# Autodesk Inventor assembly: Сборка
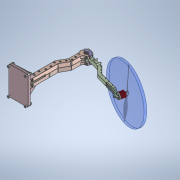
[picture p0: Inventor's stored thumbnail of the model, 180x180]
Saved by Autodesk Inventor 2021.2 (Build 252289000, 289)
## iProperties
Created: 2024-10-29
Part Number: Сборка
Document SubType Name: Assembly
Designer: barko
Mass: 1383.59 g
Surface Area: 2828.64 cm^2
Volume: 1218.78 cm^3
Density: 1.13522 g/cm^3
Author: barko
## Documents named in this file (31)
- C:\Users\DELL\Desktop\Personal\PID_controller\PID_controller\Mechanics\3D_model\Сборка.iam
- C:\Users\DELL\Desktop\Personal\PID_controller\PID_controller\Mechanics\3D_model\Детали твёрдого тела\Скобка 1.ipt
- C:\Users\DELL\Desktop\Personal\PID_controller\PID_controller\Mechanics\3D_model\Детали твёрдого тела\Скобка 2.ipt
- C:\Users\DELL\Desktop\Personal\PID_controller\PID_controller\Mechanics\3D_model\Детали твёрдого тела\Фланец.ipt
- C:\Users\DELL\Desktop\Personal\PID_controller\PID_controller\Mechanics\3D_model\Детали твёрдого тела\Луч.ipt
- C:\Users\DELL\Desktop\Personal\PID_controller\PID_controller\Mechanics\3D_model\Детали твёрдого тела\Ложечка.ipt
- C:\Users\DELL\Desktop\Personal\PID_controller\PID_controller\Mechanics\3D_model\Моторчик.ipt
- C:\Users\DELL\Desktop\Personal\PID_controller\PID_controller\Mechanics\3D_model\Пропеллер.ipt
- C:\Users\DELL\Documents\Inventor\Content Center Files\R2021\ru-RU\Nut GOST 15524-70\Гайка M4-6H ГОСТ 15524-70.ipt
- C:\Users\DELL\Documents\Inventor\Content Center Files\R2021\ru-RU\GOST 11738-84\Винт M4-6gx20 ГОСТ 11738-84.ipt
- C:\Users\DELL\Desktop\Personal\PID_controller\PID_controller\Mechanics\3D_model\Подшипник.ipt
- C:\Users\DELL\Documents\Inventor\Content Center Files\R2021\ru-RU\GOST 5915-70\Гайка M6-6H ГОСТ 5915-70(1).ipt
- C:\Users\DELL\Documents\Inventor\Content Center Files\R2021\ru-RU\GOST 11738-84\Винт M6-6gx50 ГОСТ 11738-84.ipt
- C:\Users\DELL\Documents\Inventor\Content Center Files\R2021\ru-RU\GOST 11371-78  A\Шайба 6 ГОСТ 11371-78.ipt
- C:\Users\DELL\Documents\Inventor\Content Center Files\R2021\ru-RU\Washer 1 GOST 6402-78\Шайба 6Л ГОСТ 6402-78.ipt
- C:\Users\DELL\Documents\Inventor\Content Center Files\R2021\ru-RU\GOST 17475-80 (2)\Винт 2.M6-6gx30 ГОСТ 17475-80.ipt
- C:\Users\DELL\Documents\Inventor\Content Center Files\R2021\ru-RU\ISO 10642(1)\ISO 10642 - M3x8.ipt
- C:\Users\DELL\Documents\Inventor\Content Center Files\R2021\ru-RU\ISO 10642(1)\ISO 10642 - M3x12.ipt
- C:\Users\DELL\Desktop\Personal\PID_controller\PID_controller\Mechanics\3D_model\Детали твёрдого тела\Вал насадка 1.ipt
- C:\Users\DELL\Desktop\Personal\PID_controller\PID_controller\Mechanics\3D_model\Метизы\Шайба A 4 ГОСТ 6958-78.ipt
- C:\Users\DELL\Documents\Inventor\Content Center Files\R2021\ru-RU\GOST 5916-70\Гайка M4-6H ГОСТ 5916-70.ipt
- C:\Users\DELL\Documents\Inventor\Content Center Files\R2021\ru-RU\GOST 11738-84\Винт M4-6gx25 ГОСТ 11738-84.ipt
- C:\Users\DELL\Documents\Inventor\Content Center Files\R2021\ru-RU\GOST 11738-84\Винт M6-6gx30 ГОСТ 11738-84.ipt
- C:\Users\DELL\Desktop\Personal\PID_controller\PID_controller\Mechanics\3D_model\Детали твёрдого тела\Блок.ipt
- C:\Users\DELL\Desktop\Personal\PID_controller\PID_controller\Mechanics\3D_model\Детали твёрдого тела\Ножка левая верх.ipt
- C:\Users\DELL\Desktop\Personal\PID_controller\PID_controller\Mechanics\3D_model\Детали твёрдого тела\Ножка левая низ.ipt
- C:\Users\DELL\Desktop\Personal\PID_controller\PID_controller\Mechanics\3D_model\Детали твёрдого тела\Ножка правая верх.ipt
- C:\Users\DELL\Desktop\Personal\PID_controller\PID_controller\Mechanics\3D_model\Детали твёрдого тела\Ножка правая низ.ipt
- C:\Users\DELL\Documents\Inventor\Content Center Files\R2021\ru-RU\GOST 11738-84\Винт M4-6gx30 ГОСТ 11738-84.ipt
- C:\Users\DELL\Desktop\Personal\PID_controller\PID_controller\Mechanics\3D_model\Метизы\Винт M3-6gx8 ГОСТ 11738-84.ipt
- C:\Users\DELL\Desktop\Personal\PID_controller\PID_controller\Mechanics\3D_model\Метизы\Винт M4-6gx40 ГОСТ 1491-80.ipt
## Components (78 placed, 30 different names)
1. Скобка 1:1 — Совмещение:104, Совмещение:109
2. Скобка 2:1 — Совмещение:119, Совмещение:120
3. Фланец:1 — Вставка:6, Вставка:7, Вставка:8, Вставка:9, Заподлицо:2, Заподлицо:3, Заподлицо:4, Заподлицо:5, Совмещение:127, Совмещение:128, Совмещение:129, Совмещение:130, Совмещение:131, Совмещение:132, Совмещение:133, Совмещение:134, Совмещение:135, Совмещение:136, Совмещение:137, Совмещение:138
4. Луч:1 — Заподлицо:1, Совмещение:96, Совмещение:97, Заподлицо:6, Совмещение:111, Совмещение:112, Совмещение:114, Совмещение:199
5. Ложечка:1 — Совмещение:87, Совмещение:88, Совмещение:91, Совмещение:92, Совмещение:93, Совмещение:94, Совмещение:96, Совмещение:97, Заподлицо:6, Совмещение:98, Совмещение:99, Вставка:37
6. Моторчик:1 — Вставка:2, Совмещение:98, Совмещение:99
7. Пропеллер:1 — Вставка:2
8. Подшипник:1 — Вставка:25, Вставка:29, Вставка:39
9. Подшипник:2 — Вставка:32, Вставка:34
10. Вал насадка 1:1 — Вставка:25, Вставка:32, Совмещение:199
11. Шайба A 4 ГОСТ 6958-78:3 — Вставка:29, Вставка:38
12. Блок:1
13. Шайба A 4 ГОСТ 6958-78:4 — Вставка:34, Вставка:36
14. Гайка ГОСТ 15524-70 M4:7 — Вставка:36
15. Ножка левая верх:1 — Совмещение:152, Совмещение:153, Совмещение:154, Совмещение:155, Совмещение:156, Совмещение:157, Совмещение:213, Совмещение:215, Совмещение:231, Совмещение:233, Совмещение:235, Совмещение:237, Совмещение:239, Совмещение:241, Совмещение:243
16. Ножка левая низ:1 — Совмещение:143, Совмещение:145
17. Ножка правая верх:1 — Совмещение:147, Совмещение:148, Совмещение:149, Совмещение:150, Совмещение:151, Совмещение:158, Вставка:39, Совмещение:208, Совмещение:209, Совмещение:210, Совмещение:211, Совмещение:212, Совмещение:214
18. Ножка правая низ:1 — Совмещение:144, Совмещение:146, Совмещение:216, Совмещение:217, Совмещение:218, Совмещение:219, Совмещение:220, Совмещение:221, Совмещение:222, Совмещение:223, Совмещение:224, Совмещение:225, Совмещение:226, Совмещение:227, Совмещение:228, Совмещение:229, Совмещение:230, Совмещение:232, Совмещение:234, Совмещение:236, Совмещение:238, Совмещение:240, Совмещение:242
19. Винт M4-6gx40 ГОСТ 1491-80:1 — Вставка:38
20. Винт ГОСТ 11738-84 M 4x30:4 — Совмещение:216, Совмещение:217
21. Гайка ГОСТ 5916-70 M4:4 — Совмещение:230, Совмещение:231
22. Винт ГОСТ 11738-84 M 4x30:6 — Совмещение:218, Совмещение:219
23. Винт ГОСТ 11738-84 M 4x30:7 — Совмещение:220, Совмещение:221
24. Винт ГОСТ 11738-84 M 4x30:8 — Совмещение:222, Совмещение:223
25. Винт ГОСТ 11738-84 M 4x30:9 — Совмещение:224, Совмещение:225
26. Винт ГОСТ 11738-84 M 4x30:10 — Совмещение:226, Совмещение:227
27. Винт ГОСТ 11738-84 M 4x30:11 — Совмещение:228, Совмещение:229
28. Гайка ГОСТ 5916-70 M4:6 — Совмещение:232, Совмещение:233
29. Гайка ГОСТ 5916-70 M4:7 — Совмещение:234, Совмещение:235
30. Гайка ГОСТ 5916-70 M4:8 — Совмещение:236, Совмещение:237
31. Гайка ГОСТ 5916-70 M4:9 — Совмещение:238, Совмещение:239
32. Гайка ГОСТ 5916-70 M4:10 — Совмещение:240, Совмещение:241
33. Гайка ГОСТ 5916-70 M4:11 — Совмещение:242, Совмещение:243
34. Гайка ГОСТ 5916-70 M4:5 — Совмещение:214, Совмещение:215
35. Винт ГОСТ 11738-84 M 4x30:5 — Совмещение:210, Совмещение:211
36. Гайка ГОСТ 5916-70 M4:1 — Совмещение:212, Совмещение:213
37. Винт ГОСТ 11738-84 M 4x30:1 — Совмещение:208, Совмещение:209
38. Винт ГОСТ 11738-84 M 4x25:1 — Совмещение:103, Совмещение:104
39. Гайка ГОСТ 15524-70 M4:1 — Совмещение:103, Совмещение:147, Совмещение:148, Совмещение:149
40. Винт ГОСТ 11738-84 M 4x25:2 — Совмещение:113, Совмещение:114
41. Гайка ГОСТ 15524-70 M4:2 — Совмещение:111, Совмещение:112, Совмещение:113
42. Винт ГОСТ 11738-84 M 4x20:2 — Совмещение:108, Совмещение:109
43. Винт ГОСТ 11738-84 M 4x25:3 — Совмещение:118, Совмещение:119
44. Винт ГОСТ 11738-84 M 4x20:4 — Совмещение:120, Совмещение:124
45. Гайка ГОСТ 15524-70 M4:3 — Совмещение:118, Совмещение:155, Совмещение:156, Совмещение:157
46. Гайка ГОСТ 15524-70 M4:4 — Совмещение:108, Совмещение:150, Совмещение:151, Совмещение:158
47. Гайка ГОСТ 15524-70 M4:5 — Совмещение:124, Совмещение:152, Совмещение:153, Совмещение:154
48. Гайка ГОСТ 5915-70 M6:1 — Совмещение:133, Совмещение:134, Совмещение:135, Совмещение:140
49. Гайка ГОСТ 5915-70 M6:2 — Совмещение:127, Совмещение:128, Совмещение:129, Совмещение:139
50. Гайка ГОСТ 5915-70 M6:3 — Совмещение:136, Совмещение:137, Совмещение:138, Совмещение:141
51. Гайка ГОСТ 5915-70 M6:4 — Совмещение:78, Совмещение:130, Совмещение:131, Совмещение:132, Совмещение:142
52. Винт ГОСТ 11738-84 M 6x50:1 — Совмещение:141, Совмещение:146
53. Винт ГОСТ 11738-84 M 6x30:1 — Совмещение:139, Совмещение:143
54. Винт ГОСТ 11738-84 M 6x30:2 — Совмещение:78, Совмещение:142, Совмещение:144
55. Винт ГОСТ 11738-84 M 6x50:2 — Совмещение:140, Совмещение:145
56. Шайба  ГОСТ 11371-78 6,4:1 — Вставка:6, Вставка:10
57. Шайба  ГОСТ 11371-78 6,4:2 — Вставка:7, Вставка:11
58. Шайба  ГОСТ 11371-78 6,4:3 — Вставка:8, Вставка:13
59. Шайба  ГОСТ 11371-78 6,4:4 — Вставка:9, Вставка:12
60. Шайба 1 ГОСТ 6402-78 6Л:1 — Вставка:10, Вставка:16
61. Шайба 1 ГОСТ 6402-78 6Л:2 — Вставка:11, Вставка:15
62. Шайба 1 ГОСТ 6402-78 6Л:3 — Вставка:12, Вставка:17
63. Шайба 1 ГОСТ 6402-78 6Л:4 — Вставка:13, Вставка:14
64. Гайка ГОСТ 5915-70 M6:5 — Вставка:14, Совмещение:85
65. Гайка ГОСТ 5915-70 M6:6 — Вставка:15, Совмещение:84
66. Гайка ГОСТ 5915-70 M6:7 — Вставка:16, Совмещение:82
67. Гайка ГОСТ 5915-70 M6:8 — Вставка:17, Совмещение:83
68. Винт 2 ГОСТ 17475-80 M6 x 30:1 — Совмещение:82, Заподлицо:3
69. Винт 2 ГОСТ 17475-80 M6 x 30:2 — Совмещение:83, Заподлицо:2
70. Винт 2 ГОСТ 17475-80 M6 x 30:3 — Совмещение:85, Заподлицо:5
71. Винт 2 ГОСТ 17475-80 M6 x 30:4 — Совмещение:84, Заподлицо:4
72. Винт M3-6gx8 ГОСТ 11738-84:1 — Вставка:37
73. ISO 10642 M3x12:2 — Совмещение:87
74. ISO 10642 M3x12:3 — Совмещение:88
75. ISO 10642 M3x8:1 — Совмещение:91
76. ISO 10642 M3x8:2 — Совмещение:92
77. ISO 10642 M3x8:3 — Совмещение:93
78. ISO 10642 M3x8:4 — Совмещение:94
## Relationships (123: Mate 96, Insert 21, Flush 6)
- Вставка:2 [Insert] (2 mm): Моторчик:1 ↔ Пропеллер:1
- Заподлицо:1 [Flush]: Луч:1
- Совмещение:78 [Mate]: Гайка ГОСТ 5915-70 M6:4 ↔ Винт ГОСТ 11738-84 M 6x30:2
- Вставка:6 [Insert]: Фланец:1 ↔ Шайба  ГОСТ 11371-78 6,4:1
- Вставка:7 [Insert]: Фланец:1 ↔ Шайба  ГОСТ 11371-78 6,4:2
- Вставка:8 [Insert]: Фланец:1 ↔ Шайба  ГОСТ 11371-78 6,4:3
- Вставка:9 [Insert]: Фланец:1 ↔ Шайба  ГОСТ 11371-78 6,4:4
- Вставка:10 [Insert]: Шайба  ГОСТ 11371-78 6,4:1 ↔ Шайба 1 ГОСТ 6402-78 6Л:1
- Вставка:11 [Insert]: Шайба  ГОСТ 11371-78 6,4:2 ↔ Шайба 1 ГОСТ 6402-78 6Л:2
- Вставка:12 [Insert]: Шайба  ГОСТ 11371-78 6,4:4 ↔ Шайба 1 ГОСТ 6402-78 6Л:3
- Вставка:13 [Insert]: Шайба  ГОСТ 11371-78 6,4:3 ↔ Шайба 1 ГОСТ 6402-78 6Л:4
- Вставка:14 [Insert]: Шайба 1 ГОСТ 6402-78 6Л:4 ↔ Гайка ГОСТ 5915-70 M6:5
- Вставка:15 [Insert]: Шайба 1 ГОСТ 6402-78 6Л:2 ↔ Гайка ГОСТ 5915-70 M6:6
- Вставка:16 [Insert]: Шайба 1 ГОСТ 6402-78 6Л:1 ↔ Гайка ГОСТ 5915-70 M6:7
- Вставка:17 [Insert]: Шайба 1 ГОСТ 6402-78 6Л:3 ↔ Гайка ГОСТ 5915-70 M6:8
- Совмещение:82 [Mate]: Гайка ГОСТ 5915-70 M6:7 ↔ Винт 2 ГОСТ 17475-80 M6 x 30:1
- Совмещение:83 [Mate]: Гайка ГОСТ 5915-70 M6:8 ↔ Винт 2 ГОСТ 17475-80 M6 x 30:2
- Совмещение:84 [Mate]: Гайка ГОСТ 5915-70 M6:6 ↔ Винт 2 ГОСТ 17475-80 M6 x 30:4
- Совмещение:85 [Mate]: Гайка ГОСТ 5915-70 M6:5 ↔ Винт 2 ГОСТ 17475-80 M6 x 30:3
- Заподлицо:2 [Flush] (9 mm): Фланец:1 ↔ Винт 2 ГОСТ 17475-80 M6 x 30:2
- Заподлицо:3 [Flush] (9 mm): Фланец:1 ↔ Винт 2 ГОСТ 17475-80 M6 x 30:1
- Заподлицо:4 [Flush] (9 mm): Фланец:1 ↔ Винт 2 ГОСТ 17475-80 M6 x 30:4
- Заподлицо:5 [Flush] (9 mm): Фланец:1 ↔ Винт 2 ГОСТ 17475-80 M6 x 30:3
- Совмещение:87 [Mate]: Ложечка:1 ↔ ISO 10642 M3x12:2
- Совмещение:88 [Mate]: Ложечка:1 ↔ ISO 10642 M3x12:3
- Совмещение:91 [Mate]: Ложечка:1 ↔ ISO 10642 M3x8:1
- Совмещение:92 [Mate]: Ложечка:1 ↔ ISO 10642 M3x8:2
- Совмещение:93 [Mate]: Ложечка:1 ↔ ISO 10642 M3x8:3
- Совмещение:94 [Mate]: Ложечка:1 ↔ ISO 10642 M3x8:4
- Совмещение:96 [Mate]: Луч:1 ↔ Ложечка:1
- Совмещение:97 [Mate]: Луч:1 ↔ Ложечка:1
- Заподлицо:6 [Flush]: Луч:1 ↔ Ложечка:1
- Совмещение:98 [Mate]: Ложечка:1 ↔ Моторчик:1
- Совмещение:99 [Mate]: Ложечка:1 ↔ Моторчик:1
- Вставка:25 [Insert]: Подшипник:1 ↔ Вал насадка 1:1
- Совмещение:103 [Mate]: Винт ГОСТ 11738-84 M 4x25:1 ↔ Гайка ГОСТ 15524-70 M4:1
- Совмещение:104 [Mate]: Скобка 1:1 ↔ Винт ГОСТ 11738-84 M 4x25:1
- Совмещение:108 [Mate]: Винт ГОСТ 11738-84 M 4x20:2 ↔ Гайка ГОСТ 15524-70 M4:4
- Совмещение:109 [Mate]: Скобка 1:1 ↔ Винт ГОСТ 11738-84 M 4x20:2
- Совмещение:111 [Mate]: Луч:1 ↔ Гайка ГОСТ 15524-70 M4:2
- Совмещение:112 [Mate]: Луч:1 ↔ Гайка ГОСТ 15524-70 M4:2
- Совмещение:113 [Mate]: Винт ГОСТ 11738-84 M 4x25:2 ↔ Гайка ГОСТ 15524-70 M4:2
- Совмещение:114 [Mate]: Луч:1 ↔ Винт ГОСТ 11738-84 M 4x25:2
- Совмещение:118 [Mate]: Винт ГОСТ 11738-84 M 4x25:3 ↔ Гайка ГОСТ 15524-70 M4:3
- Совмещение:119 [Mate]: Скобка 2:1 ↔ Винт ГОСТ 11738-84 M 4x25:3
- Совмещение:120 [Mate]: Скобка 2:1 ↔ Винт ГОСТ 11738-84 M 4x20:4
- Совмещение:124 [Mate]: Винт ГОСТ 11738-84 M 4x20:4 ↔ Гайка ГОСТ 15524-70 M4:5
- Вставка:29 [Insert]: Подшипник:1 ↔ Шайба A 4 ГОСТ 6958-78:3
- Вставка:32 [Insert]: Подшипник:2 ↔ Вал насадка 1:1
- Вставка:34 [Insert]: Подшипник:2 ↔ Шайба A 4 ГОСТ 6958-78:4
- Вставка:36 [Insert]: Шайба A 4 ГОСТ 6958-78:4 ↔ Гайка ГОСТ 15524-70 M4:7
- Совмещение:127 [Mate]: Фланец:1 ↔ Гайка ГОСТ 5915-70 M6:2
- Совмещение:128 [Mate]: Фланец:1 ↔ Гайка ГОСТ 5915-70 M6:2
- Совмещение:129 [Mate]: Фланец:1 ↔ Гайка ГОСТ 5915-70 M6:2
- Совмещение:130 [Mate]: Фланец:1 ↔ Гайка ГОСТ 5915-70 M6:4
- Совмещение:131 [Mate]: Фланец:1 ↔ Гайка ГОСТ 5915-70 M6:4
- Совмещение:132 [Mate]: Фланец:1 ↔ Гайка ГОСТ 5915-70 M6:4
- Совмещение:133 [Mate]: Фланец:1 ↔ Гайка ГОСТ 5915-70 M6:1
- Совмещение:134 [Mate]: Фланец:1 ↔ Гайка ГОСТ 5915-70 M6:1
- Совмещение:135 [Mate]: Фланец:1 ↔ Гайка ГОСТ 5915-70 M6:1
- Совмещение:136 [Mate]: Фланец:1 ↔ Гайка ГОСТ 5915-70 M6:3
- Совмещение:137 [Mate]: Фланец:1 ↔ Гайка ГОСТ 5915-70 M6:3
- Совмещение:138 [Mate]: Фланец:1 ↔ Гайка ГОСТ 5915-70 M6:3
- Совмещение:139 [Mate]: Гайка ГОСТ 5915-70 M6:2 ↔ Винт ГОСТ 11738-84 M 6x30:1
- Совмещение:140 [Mate]: Гайка ГОСТ 5915-70 M6:1 ↔ Винт ГОСТ 11738-84 M 6x50:2
- Совмещение:141 [Mate]: Гайка ГОСТ 5915-70 M6:3 ↔ Винт ГОСТ 11738-84 M 6x50:1
- Совмещение:142 [Mate]: Гайка ГОСТ 5915-70 M6:4 ↔ Винт ГОСТ 11738-84 M 6x30:2
- Совмещение:143 [Mate]: Ножка левая низ:1 ↔ Винт ГОСТ 11738-84 M 6x30:1
- Совмещение:144 [Mate]: Ножка правая низ:1 ↔ Винт ГОСТ 11738-84 M 6x30:2
- Совмещение:145 [Mate]: Ножка левая низ:1 ↔ Винт ГОСТ 11738-84 M 6x50:2
- Совмещение:146 [Mate]: Ножка правая низ:1 ↔ Винт ГОСТ 11738-84 M 6x50:1
- Совмещение:147 [Mate]: Ножка правая верх:1 ↔ Гайка ГОСТ 15524-70 M4:1
- Совмещение:148 [Mate]: Ножка правая верх:1 ↔ Гайка ГОСТ 15524-70 M4:1
- Совмещение:149 [Mate]: Ножка правая верх:1 ↔ Гайка ГОСТ 15524-70 M4:1
- Совмещение:150 [Mate]: Ножка правая верх:1 ↔ Гайка ГОСТ 15524-70 M4:4
- Совмещение:151 [Mate]: Ножка правая верх:1 ↔ Гайка ГОСТ 15524-70 M4:4
- Совмещение:152 [Mate]: Ножка левая верх:1 ↔ Гайка ГОСТ 15524-70 M4:5
- Совмещение:153 [Mate]: Ножка левая верх:1 ↔ Гайка ГОСТ 15524-70 M4:5
- Совмещение:154 [Mate]: Ножка левая верх:1 ↔ Гайка ГОСТ 15524-70 M4:5
- Совмещение:155 [Mate]: Ножка левая верх:1 ↔ Гайка ГОСТ 15524-70 M4:3
- Совмещение:156 [Mate]: Ножка левая верх:1 ↔ Гайка ГОСТ 15524-70 M4:3
- Совмещение:157 [Mate]: Ножка левая верх:1 ↔ Гайка ГОСТ 15524-70 M4:3
- Совмещение:158 [Mate]: Ножка правая верх:1 ↔ Гайка ГОСТ 15524-70 M4:4
- Вставка:37 [Insert]: Ложечка:1 ↔ Винт M3-6gx8 ГОСТ 11738-84:1
- Вставка:38 [Insert]: Шайба A 4 ГОСТ 6958-78:3 ↔ Винт M4-6gx40 ГОСТ 1491-80:1
- Вставка:39 [Insert]: Подшипник:1 ↔ Ножка правая верх:1
- Совмещение:199 [Mate]: Луч:1 ↔ Вал насадка 1:1
- Совмещение:208 [Mate]: Ножка правая верх:1 ↔ Винт ГОСТ 11738-84 M 4x30:1
- Совмещение:209 [Mate]: Ножка правая верх:1 ↔ Винт ГОСТ 11738-84 M 4x30:1
- Совмещение:210 [Mate]: Ножка правая верх:1 ↔ Винт ГОСТ 11738-84 M 4x30:5
- Совмещение:211 [Mate]: Ножка правая верх:1 ↔ Винт ГОСТ 11738-84 M 4x30:5
- Совмещение:212 [Mate]: Ножка правая верх:1 ↔ Гайка ГОСТ 5916-70 M4:1
- Совмещение:213 [Mate]: Ножка левая верх:1 ↔ Гайка ГОСТ 5916-70 M4:1
- Совмещение:214 [Mate]: Ножка правая верх:1 ↔ Гайка ГОСТ 5916-70 M4:5
- Совмещение:215 [Mate]: Ножка левая верх:1 ↔ Гайка ГОСТ 5916-70 M4:5
- Совмещение:216 [Mate]: Ножка правая низ:1 ↔ Винт ГОСТ 11738-84 M 4x30:4
- Совмещение:217 [Mate]: Ножка правая низ:1 ↔ Винт ГОСТ 11738-84 M 4x30:4
- Совмещение:218 [Mate]: Ножка правая низ:1 ↔ Винт ГОСТ 11738-84 M 4x30:6
- Совмещение:219 [Mate]: Ножка правая низ:1 ↔ Винт ГОСТ 11738-84 M 4x30:6
- Совмещение:220 [Mate]: Ножка правая низ:1 ↔ Винт ГОСТ 11738-84 M 4x30:7
- Совмещение:221 [Mate]: Ножка правая низ:1 ↔ Винт ГОСТ 11738-84 M 4x30:7
- Совмещение:222 [Mate]: Ножка правая низ:1 ↔ Винт ГОСТ 11738-84 M 4x30:8
- Совмещение:223 [Mate]: Ножка правая низ:1 ↔ Винт ГОСТ 11738-84 M 4x30:8
- Совмещение:224 [Mate]: Ножка правая низ:1 ↔ Винт ГОСТ 11738-84 M 4x30:9
- Совмещение:225 [Mate]: Ножка правая низ:1 ↔ Винт ГОСТ 11738-84 M 4x30:9
- Совмещение:226 [Mate]: Ножка правая низ:1 ↔ Винт ГОСТ 11738-84 M 4x30:10
- Совмещение:227 [Mate]: Ножка правая низ:1 ↔ Винт ГОСТ 11738-84 M 4x30:10
- Совмещение:228 [Mate]: Ножка правая низ:1 ↔ Винт ГОСТ 11738-84 M 4x30:11
- Совмещение:229 [Mate]: Ножка правая низ:1 ↔ Винт ГОСТ 11738-84 M 4x30:11
- Совмещение:230 [Mate]: Ножка правая низ:1 ↔ Гайка ГОСТ 5916-70 M4:4
- Совмещение:231 [Mate]: Ножка левая верх:1 ↔ Гайка ГОСТ 5916-70 M4:4
- Совмещение:232 [Mate]: Ножка правая низ:1 ↔ Гайка ГОСТ 5916-70 M4:6
- Совмещение:233 [Mate]: Ножка левая верх:1 ↔ Гайка ГОСТ 5916-70 M4:6
- Совмещение:234 [Mate]: Ножка правая низ:1 ↔ Гайка ГОСТ 5916-70 M4:7
- Совмещение:235 [Mate]: Ножка левая верх:1 ↔ Гайка ГОСТ 5916-70 M4:7
- Совмещение:236 [Mate]: Ножка правая низ:1 ↔ Гайка ГОСТ 5916-70 M4:8
- Совмещение:237 [Mate]: Ножка левая верх:1 ↔ Гайка ГОСТ 5916-70 M4:8
- Совмещение:238 [Mate]: Ножка правая низ:1 ↔ Гайка ГОСТ 5916-70 M4:9
- Совмещение:239 [Mate]: Ножка левая верх:1 ↔ Гайка ГОСТ 5916-70 M4:9
- Совмещение:240 [Mate]: Ножка правая низ:1 ↔ Гайка ГОСТ 5916-70 M4:10
- Совмещение:241 [Mate]: Ножка левая верх:1 ↔ Гайка ГОСТ 5916-70 M4:10
- Совмещение:242 [Mate]: Ножка правая низ:1 ↔ Гайка ГОСТ 5916-70 M4:11
- Совмещение:243 [Mate]: Ножка левая верх:1 ↔ Гайка ГОСТ 5916-70 M4:11
